# Autodesk Inventor assembly: Pump_Total
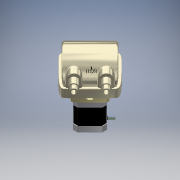
[picture p0: Inventor's stored thumbnail of the model, 180x180]
Saved by Autodesk Inventor 2016 (Build 200138000, 138)
## iProperties
Created: 2015-06-30
Part Number: Pump_Total
Document SubType Name: Assembly
Designer: bastli
Mass: 829.915 g
Surface Area: 587.932 cm^2
Volume: 273.34 cm^3
Density: 3.0362 g/cm^3
Author: bastli
## Documents named in this file (5)
- C:\Users\3DPrinterUser\Documents\GitHub\BarBot\Conception\Mechanical\Pump_Block\Pump_Total.iam
- C:\Users\3DPrinterUser\Documents\GitHub\BarBot\Conception\Mechanical\Pump_Block\Pump_Head.ipt
- C:\Users\3DPrinterUser\Documents\GitHub\BarBot\Conception\Mechanical\Pump_Block\M1173041- NEMA 17.ipt
- C:\Users\3DPrinterUser\Documents\GitHub\BarBot\Conception\Mechanical\Pump_Block\Pump_Adapter.ipt
- C:\Users\3DPrinterUser\Documents\GitHub\BarBot\Conception\Mechanical\Pump_Block\Honlite Axes Adapter.ipt
## Components (4 placed, 4 different names)
1. Pump_Head:1 — Rigid:2
2. M1173041- NEMA 17:1 — Rotational:1, Rotational:2
3. Honlite Axes Adapter:1 — Rotational:1
4. Pump_Adapter:1 — Rigid:2, Rotational:2
## Relationships (3: RevoluteJoint 2, WeldJoint 1)
- Rigid:2 [WeldJoint]: Pump_Head:1 ↔ Pump_Adapter:1
- Rotational:1 [RevoluteJoint]: M1173041- NEMA 17:1 ↔ Honlite Axes Adapter:1
- Rotational:2 [RevoluteJoint]: M1173041- NEMA 17:1 ↔ Pump_Adapter:1
## Named parameters: Axis_Stop_Offset = 12.3 mm, Axis_Adapter_Length = 34.78884 mm
